# Autodesk Inventor assembly: 000.003 - Блок АКБ СБ
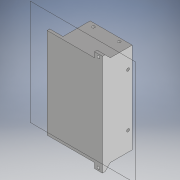
[picture p0: Inventor's stored thumbnail of the model, 180x180]
Saved by Autodesk Inventor 2022 (Build 260153000, 153)
## iProperties
Created: 2022-02-26
Part Number: 000.003 - Блок АКБ СБ
Document SubType Name: Assembly
Designer: Petrov Ivan
Author: Petrov Ivan
## Documents named in this file (3)
- C:\Users\Ivan Petrov\Documents\GitHub\OmniBot\design\000.003 - Блок АКБ СБ.iam
- C:\Users\Ivan Petrov\Documents\GitHub\OmniBot\design\000.003.001 - Основание.ipt
- C:\Users\Ivan Petrov\Documents\GitHub\OmniBot\design\standart_components\NUCLEO.ipt
## Components (3 placed, 2 different names)
1. 000.003.001 - Основание.ipt:1 — Касательность:1, Угол:1, Касательность:2, Заподлицо:1
2. NUCLEO.ipt:1 — Касательность:1, Угол:1, Совмещение:1, Заподлицо:1
3. NUCLEO.ipt:2 — Совмещение:1, Касательность:2
## Relationships (5: Tangent 2, Angle 1, Mate 1, Flush 1)
- Касательность:1 [Tangent]: 000.003.001 - Основание.ipt:1 ↔ NUCLEO.ipt:1
- Угол:1 [Angle] (0 deg): 000.003.001 - Основание.ipt:1 ↔ NUCLEO.ipt:1
- Совмещение:1 [Mate] (10 mm): NUCLEO.ipt:1 ↔ NUCLEO.ipt:2
- Касательность:2 [Tangent]: 000.003.001 - Основание.ipt:1 ↔ NUCLEO.ipt:2
- Заподлицо:1 [Flush] (20 mm): 000.003.001 - Основание.ipt:1 ↔ NUCLEO.ipt:1
